# Autodesk Inventor assembly: Chuck with Baseplate Staging Plate
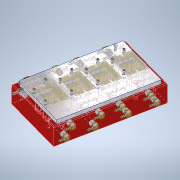
[picture p0: Inventor's stored thumbnail of the model, 180x180]
Saved by Autodesk Inventor 2022 (Build 260153000, 153)
## iProperties
Created: 2021-11-30
Part Number: Chuck with Baseplate Staging Plate
Document SubType Name: Assembly
Designer: Caleb
Author: Caleb
## Documents named in this file (3)
- C:\Users\Caleb\Desktop\nebraska-silicon-lab\Hardware\ETL\Module Assembly\Chuck - 16-pocket V1\Chuck with Baseplate Staging Plate.iam
- C:\Users\Caleb\Desktop\nebraska-silicon-lab\Hardware\ETL\Module Assembly\Chuck - 16-pocket V1\Chuck - 16-pocket.iam
- C:\Users\Caleb\Desktop\nebraska-silicon-lab\Hardware\ETL\Module Assembly\Baseplate Staging Plate - V1\Baseplate Staging Plate Assembly - V1.iam
## Components (2 placed, 2 different names)
1. Chuck - 16-pocket:1 [sub-assembly] — Mate:1, Angle:1, Tangent:1, Tangent:2
2. Baseplate Staging Plate Assembly - V1:1 [sub-assembly] — Mate:1, Angle:1, Tangent:1, Tangent:2
## Relationships (4: Tangent 2, Mate 1, Angle 1)
- Mate:1: Chuck - 16-pocket:1 ↔ Baseplate Staging Plate Assembly - V1:1
- Angle:1 (0 deg): Chuck - 16-pocket:1 ↔ Baseplate Staging Plate Assembly - V1:1
- Tangent:1: Chuck - 16-pocket:1 ↔ Baseplate Staging Plate Assembly - V1:1
- Tangent:2: Chuck - 16-pocket:1 ↔ Baseplate Staging Plate Assembly - V1:1
